# Autodesk Inventor assembly: Toughbox-mini-hex-long
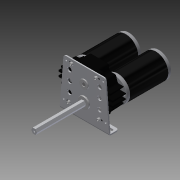
[picture p0: Inventor's stored thumbnail of the model, 180x180]
Saved by Autodesk Inventor 2013 (Build 170138000, 138)
## iProperties
Created: 2013-01-13
Part Number: Toughbox-mini-hex-long
Document SubType Name: Assembly
Designer: Moses
Mass: 3524.5 g
Surface Area: 2045.83 cm^2
Volume: 988.828 cm^3
Density: 3.56432 g/cm^3
Translation Standard: STEP AP203
FileName: S:/Products/Gearboxes Spur Single Stage/Toughbox/Toughbox Mini/Toughbox-Mini.stp
PreProcessor: Unknown
PostProcessor: Build: 138, Release: 2013 RTM - Date: Thu 03/01/2012
Sent Units: millimeter
Uncertainty: 0.001
Author: Moses
## Documents named in this file (17)
- C:\Users\Arpan\Documents\GitHub\frc2013CAD\Drivetrain\Toughbox-mini\Toughbox-mini-hex-long.iam
- C:\Users\Arpan\Documents\GitHub\frc2013CAD\Drivetrain\Toughbox-mini\r6zz.ipt
- C:\Users\Arpan\Documents\GitHub\frc2013CAD\Drivetrain\Toughbox-mini\Toughbox_d07.ipt
- C:\Users\Arpan\Documents\GitHub\frc2013CAD\Drivetrain\Toughbox-mini\Toughbox_d05.ipt
- C:\Users\Arpan\Documents\GitHub\frc2013CAD\Drivetrain\Toughbox-mini\Toughbox_d08.ipt
- C:\Users\Arpan\Documents\GitHub\frc2013CAD\Drivetrain\Toughbox-mini\Toughbox_d06.ipt
- C:\Users\Arpan\Documents\GitHub\frc2013CAD\Drivetrain\Toughbox-mini\fr-6-zz.ipt
- C:\Users\Arpan\Documents\GitHub\frc2013CAD\Drivetrain\Toughbox-mini\10-32_nylock_nut.ipt
- C:\Users\Arpan\Documents\GitHub\frc2013CAD\Drivetrain\Toughbox-mini\5-16_washer.ipt
- C:\Users\Arpan\Documents\GitHub\frc2013CAD\Drivetrain\Toughbox-mini\Toughbox_d09.ipt
- C:\Users\Arpan\Documents\GitHub\frc2013CAD\Drivetrain\Toughbox-mini\8mm_spring_clip.ipt
- C:\Users\Arpan\Documents\GitHub\frc2013CAD\Drivetrain\Toughbox-mini\Toughbox-mini_d01-5-12.ipt
- C:\Users\Arpan\Documents\GitHub\frc2013CAD\Drivetrain\Toughbox-mini\Toughbox-mini_d02.ipt
- C:\Users\Arpan\Documents\GitHub\frc2013CAD\Drivetrain\Toughbox-mini\10-32x0625_shcs.ipt
- C:\Users\Arpan\Documents\GitHub\frc2013CAD\Drivetrain\Toughbox-mini\CIM motor1.ipt
- C:\Users\Arpan\Documents\GitHub\frc2013CAD\Drivetrain\Toughbox-mini\Toughbox_d31.ipt
- C:\Users\Arpan\Documents\GitHub\frc2013CAD\Drivetrain\Toughbox-mini\fr8zz-hex.ipt
## Components (33 placed, 16 different names)
1. r6zz:1
2. r6zz:2 — Mate:2, Mate:1
3. Toughbox_d31:1 — Mate:1, Mate:2
4. Toughbox_d07:1
5. Toughbox_d05:1
6. Toughbox_d08:1
7. Toughbox_d06:1
8. fr-6-zz:1
9. fr8zz-hex:1 — Insert:3
10. 10-32_nylock_nut:1
11. 10-32_nylock_nut:2
12. 10-32_nylock_nut:3 — Insert:9
13. 10-32_nylock_nut:4 — Insert:8
14. 5-16_washer:1
15. 5-16_washer:2
16. 5-16_washer:3
17. 5-16_washer:4
18. Toughbox_d09:1
19. Toughbox_d09:2
20. 8mm_spring_clip:1
21. 8mm_spring_clip:2
22. Toughbox-mini_d01-5-12:1 — Insert:1, Insert:2, Insert:8, Insert:9
23. Toughbox-mini_d02:1 — Insert:3, Insert:4, Insert:5, Insert:6, Insert:7
24. 10-32x0625_shcs:1
25. 10-32x0625_shcs:2 — Insert:5
26. 10-32x0625_shcs:3 — Insert:6
27. 10-32x0625_shcs:4 — Insert:7
28. 10-32x0625_shcs:5 — Insert:4
29. 10-32x0625_shcs:6
30. 10-32x0625_shcs:7
31. 10-32x0625_shcs:8
32. CIM motor1:1 — Insert:1
33. CIM motor1:2 — Insert:2
## Relationships (11: Insert 9, Mate 2)
- Insert:1: Toughbox-mini_d01-5-12:1 ↔ CIM motor1:1
- Insert:2: Toughbox-mini_d01-5-12:1 ↔ CIM motor1:2
- Mate:1: r6zz:2 ↔ Toughbox_d31:1
- Mate:2: r6zz:2 ↔ Toughbox_d31:1
- Insert:3: fr8zz-hex:1 ↔ Toughbox-mini_d02:1
- Insert:4: Toughbox-mini_d02:1 ↔ 10-32x0625_shcs:5
- Insert:5: Toughbox-mini_d02:1 ↔ 10-32x0625_shcs:2
- Insert:6: Toughbox-mini_d02:1 ↔ 10-32x0625_shcs:3
- Insert:7: Toughbox-mini_d02:1 ↔ 10-32x0625_shcs:4
- Insert:8: 10-32_nylock_nut:4 ↔ Toughbox-mini_d01-5-12:1
- Insert:9: 10-32_nylock_nut:3 ↔ Toughbox-mini_d01-5-12:1
